# Autodesk Inventor assembly: motor
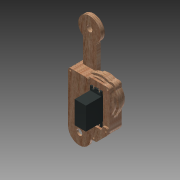
[picture p0: Inventor's stored thumbnail of the model, 180x180]
Saved by Autodesk Inventor 2015 (Build 190159000, 159)
## iProperties
Created: 2016-02-03
Part Number: motor
Document SubType Name: Assembly
Designer: david
Author: david
## Documents named in this file (11)
- Z:\gip\Inventor\generatie 7\motor v2\motor.iam
- Z:\gip\Inventor\generatie 7\motor v2\p1.ipt
- Z:\gip\Inventor\generatie 7\motor v2\p2.ipt
- Z:\gip\Inventor\generatie 7\motor v2\p3.ipt
- Z:\gip\Inventor\generatie 7\motor v2\servo\tang.ipt
- Z:\gip\Inventor\generatie 7\motor v2\p5.ipt
- Z:\gip\Inventor\generatie 7\motor v2\servo\block.ipt
- Z:\gip\Inventor\generatie 7\motor v2\tandwiel\tandwiel.iam
- Z:\gip\Inventor\generatie 7\old\Motor\tanden2.ipt
- Z:\gip\Inventor\generatie 7\motor v2\p6.ipt
- Z:\gip\Inventor\generatie 7\motor v2\p5 big.ipt
## Components (13 placed, 10 different names)
1. p1:1 — Mate:1, Flush:2, Flush:4, Flush:16, Flush:18
2. p2:1 — Mate:1, Flush:2, Mate:2, Flush:5, Mate:22
3. p2:2 — Mate:2, Flush:4, Mate:3, Mate:15, Mate:21, Mate:22, Flush:16, Mate:23, Flush:20
4. p3:1 — Mate:3, Flush:5, Mate:13, Mate:23, Mate:32, Mate:33
5. p5:2 — Flush:18, Mate:29, Mate:30, Mate:31, Mate:38, Mate:39, Flush:25, Flush:26, Mate:42, Mate:44
6. block:1 — Mate:10, Mate:11, Mate:29, Mate:30, Mate:31
7. tang:1 — Mate:10, Mate:11, Mate:18, Mate:43
8. tanden2:1 — Mate:13, Mate:15, Rotation/Translation:1, Mate:19, Flush:13, Mate:20
9. tandwiel:1 [sub-assembly] — Mate:18, Rotation/Translation:1, Flush:19, Mate:43
10. tanden2:2 — Mate:19, Flush:13, Mate:20, Mate:21, Flush:19
11. p3:2 — Mate:32, Flush:20, Mate:33, Mate:41, Flush:23, Flush:24, Flush:25
12. p5 big:1 — Mate:41, Flush:23, Flush:24, Flush:26, Mate:42
13. p6:1 — Mate:38, Mate:39, Mate:44
## Relationships (37: Mate 24, Flush 12, RelateRotateTranslate 1)
- Mate:1: p1:1 ↔ p2:1
- Flush:2: p1:1 ↔ p2:1
- Mate:2: p2:1 ↔ p2:2
- Flush:4: p1:1 ↔ p2:2
- Mate:3: p2:2 ↔ p3:1
- Flush:5: p2:1 ↔ p3:1
- Mate:10: block:1 ↔ tang:1
- Mate:11: block:1 ↔ tang:1
- Mate:13: p3:1 ↔ tanden2:1
- Mate:15: p2:2 ↔ tanden2:1
- Mate:18: tang:1 ↔ tandwiel:1
- Rotation/Translation:1 [RelateRotateTranslate] (100 mm): tanden2:1 ↔ tandwiel:1
- Mate:19: tanden2:1 ↔ tanden2:2
- Flush:13: tanden2:1 ↔ tanden2:2
- Mate:20: tanden2:1 ↔ tanden2:2
- Mate:21: p2:2 ↔ tanden2:2
- Mate:22: p2:1 ↔ p2:2
- Flush:16: p1:1 ↔ p2:2
- Mate:23: p2:2 ↔ p3:1
- Flush:18: p1:1 ↔ p5:2
- Mate:29: p5:2 ↔ block:1
- Mate:30: p5:2 ↔ block:1
- Mate:31: p5:2 ↔ block:1
- Flush:19: tandwiel:1 ↔ tanden2:2
- Mate:32: p3:1 ↔ p3:2
- Flush:20: p2:2 ↔ p3:2
- Mate:33: p3:1 ↔ p3:2
- Mate:38: p5:2 ↔ p6:1
- Mate:39: p5:2 ↔ p6:1
- Mate:41: p3:2 ↔ p5 big:1
- Flush:23: p3:2 ↔ p5 big:1
- Flush:24: p3:2 ↔ p5 big:1
- Flush:25: p5:2 ↔ p3:2
- Flush:26: p5:2 ↔ p5 big:1
- Mate:42: p5:2 ↔ p5 big:1
- Mate:43: tang:1 ↔ tandwiel:1
- Mate:44: p5:2 ↔ p6:1
